# Autodesk Inventor assembly: XY Joint Right
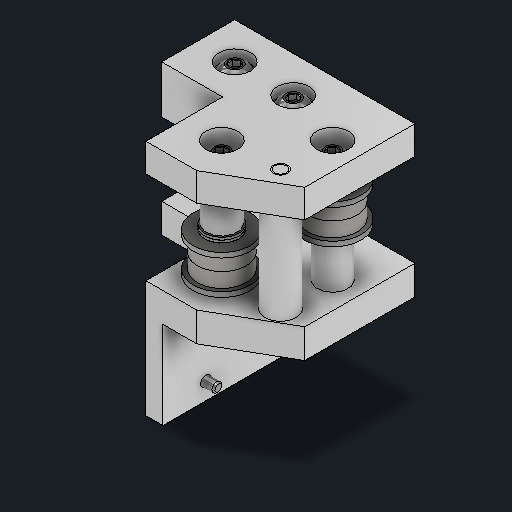
[picture p0: Inventor's stored thumbnail of the model, 512x512]
Saved by Autodesk Inventor 2025.1 (Build 291241020, 241B)
## iProperties
Created: 2025-05-09
Part Number: XY Joint Right
Document SubType Name: Assembly
Designer: AdminForWorker
Title: XY Joint Right
Author: AdminForWorker
## Documents named in this file (9)
- C:\Users\Joshua Eah\Documents\Voron 0.2\CAD\Master Assembly\X Axis\XY Joint Right.iam
- C:\Users\Joshua Eah\Documents\Voron 0.2\CAD\Machined Parts\XY Joints\XY Joint Right\XY Joint Right.iam
- C:\Users\Joshua Eah\Documents\Voron 0.2\CAD\Master Assembly\Hardware\M3x25 BHCS.ipt
- C:\Users\Joshua Eah\Documents\Voron 0.2\CAD\Master Assembly\Hardware\M2x6 FHCS.ipt
- C:\Users\Joshua Eah\Documents\Voron 0.2\CAD\Master Assembly\Hardware\M3x12 BHCS.ipt
- C:\Users\Joshua Eah\Documents\Voron 0.2\CAD\Master Assembly\Hardware\M3x6 BHCS.ipt
- C:\Users\Joshua Eah\Documents\Voron 0.2\CAD\Master Assembly\Hardware\M3 Hexnut.ipt
- C:\Users\Joshua Eah\Documents\Voron 0.2\CAD\Master Assembly\Hardware\F623 Stack.iam
- C:\Users\Joshua Eah\Documents\Voron 0.2\CAD\Master Assembly\Hardware\M3_Washer.ipt
## Components (19 placed, 8 different names)
1. XY Joint Right:1 [sub-assembly] — Insert:1, Insert:2, Insert:3, Insert:4
2. M3x25 BHCS:3
3. M3x25 BHCS:4
4. M2x6 FHCS:5 — Insert:1
5. M2x6 FHCS:6 — Insert:4
6. M2x6 FHCS:7 — Insert:3
7. M2x6 FHCS:8 — Insert:2
8. M3x12 BHCS:1
9. M3x12 BHCS:2
10. M3x6 BHCS:1
11. M3 Hexnut:1
12. M3 Hexnut:2
13. M3 Hexnut:3
14. F623 Stack:1 [sub-assembly]
15. F623 Stack:2 [sub-assembly]
16. M3_Washer:1
17. M3_Washer:2
18. M3_Washer:3
19. M3_Washer:4
## Relationships (4: Insert 4)
- Insert:1: XY Joint Right:1 ↔ M2x6 FHCS:5
- Insert:2: XY Joint Right:1 ↔ M2x6 FHCS:8
- Insert:3: XY Joint Right:1 ↔ M2x6 FHCS:7
- Insert:4: XY Joint Right:1 ↔ M2x6 FHCS:6
